# Autodesk Inventor assembly: B_Legs0
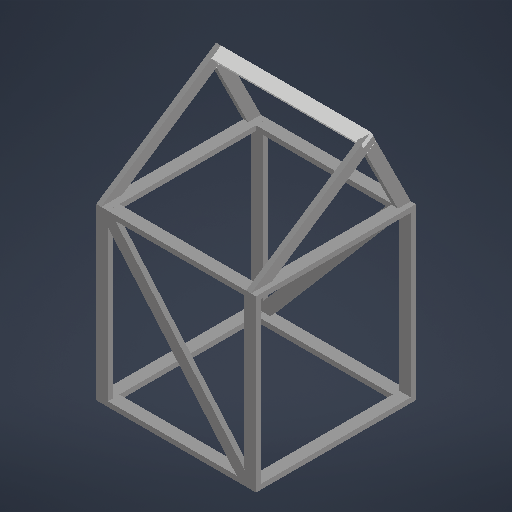
[picture p0: Inventor's stored thumbnail of the model, 512x512]
Saved by Autodesk Inventor 2026 (Build 300175000, 175)
## iProperties
Created: 2024-09-19
Part Number: B_Legs0
Document SubType Name: Assembly
Designer: User
Author: User
## Documents named in this file (8)
- C:\Users\trott\Documents\UofSC-ASME-Tiger-Burn-Design-2025\CAD\Legs\Back Leg\B_Leg.iam
- C:\Users\trott\Documents\UofSC-ASME-Tiger-Burn-Design-2025\CAD\Legs\Back Leg\2x4x96.ipt
- C:\Users\trott\Documents\UofSC-ASME-Tiger-Burn-Design-2025\CAD\Legs\Back Leg\2x4x42.ipt
- C:\Users\trott\Documents\UofSC-ASME-Tiger-Burn-Design-2025\CAD\Legs\Back Leg\2x4x48.ipt
- C:\Users\trott\Documents\UofSC-ASME-Tiger-Burn-Design-2025\CAD\Legs\Back Leg\S_2x4x44.ipt
- C:\Users\trott\Documents\UofSC-ASME-Tiger-Burn-Design-2025\CAD\Legs\Back Leg\2x4x45.ipt
- C:\Users\trott\Documents\UofSC-ASME-Tiger-Burn-Design-2025\CAD\Legs\Back Leg\S_2x4x43.267.ipt
- C:\Users\trott\Documents\UofSC-ASME-Tiger-Burn-Design-2025\CAD\Legs\Back Leg\S_2x4x23.306.ipt
## Components (19 placed, 7 different names)
1. 2x4x96:1 — Flush:1, Flush:2, Flush:3, Flush:4, Flush:5, Flush:8, Mate:3, Flush:10, Flush:12, Flush:13, Flush:14
2. 2x4x96:2 — Mate:1, Flush:1, Flush:2, Flush:3, Mate:2, Flush:6, Flush:7, Mate:5, Flush:9, Flush:11, Flush:15, Flush:16
3. 2x4x42:1 — Flush:4, Flush:5
4. 2x4x42:2 — Mate:2, Flush:6, Flush:7, Mate:4
5. 2x4x48:1 — Flush:8, Flush:13, Flush:14, Mate:7, Flush:17, Flush:20, Flush:29
6. 2x4x48:2 — Mate:5, Flush:15, Flush:16, Mate:6, Flush:18, Flush:19, Flush:27
7. 2x4x48:3 — Mate:4, Flush:9, Flush:11
8. 2x4x48:4 — Mate:3, Flush:10, Flush:12, Mate:13, Flush:28
9. 2x4x96:3 — Mate:7, Flush:17, Flush:20, Mate:8, Mate:9, Flush:23, Flush:24, Flush:29, Flush:33, Mate:19, Flush:34
10. 2x4x96:4 — Mate:6, Flush:18, Flush:19, Flush:21, Flush:22
11. 2x4x42:3 — Mate:8, Flush:21, Flush:22, Mate:12
12. 2x4x42:4 — Mate:9, Flush:23, Flush:24, Mate:18
13. S_2x4x44:1 — Flush:27
14. S_2x4x44:2 — Mate:12, Mate:13, Flush:28
15. 2x4x45:1
16. S_2x4x43.267:1 — Mate:19, Flush:34
17. S_2x4x23.306:1 — Flush:33, Mate:18
18. S_2x4x43.267:2
19. S_2x4x23.306:2
## Relationships (42: Flush 29, Mate 13)
- Mate:1: 2x4x96:2
- Flush:1: 2x4x96:1 ↔ 2x4x96:2
- Flush:2 (1130.3 mm): 2x4x96:1 ↔ 2x4x96:2
- Flush:3: 2x4x96:1 ↔ 2x4x96:2
- Flush:4: 2x4x96:1 ↔ 2x4x42:1
- Flush:5: 2x4x96:1 ↔ 2x4x42:1
- Mate:2: 2x4x96:2 ↔ 2x4x42:2
- Flush:6: 2x4x96:2 ↔ 2x4x42:2
- Flush:7: 2x4x96:2 ↔ 2x4x42:2
- Flush:8: 2x4x96:1 ↔ 2x4x48:1
- Mate:3: 2x4x96:1 ↔ 2x4x48:4
- Mate:4: 2x4x42:2 ↔ 2x4x48:3
- Mate:5: 2x4x96:2 ↔ 2x4x48:2
- Flush:9: 2x4x96:2 ↔ 2x4x48:3
- Flush:10: 2x4x96:1 ↔ 2x4x48:4
- Flush:11: 2x4x96:2 ↔ 2x4x48:3
- Flush:12: 2x4x96:1 ↔ 2x4x48:4
- Flush:13: 2x4x96:1 ↔ 2x4x48:1
- Flush:14: 2x4x96:1 ↔ 2x4x48:1
- Flush:15: 2x4x96:2 ↔ 2x4x48:2
- Flush:16: 2x4x96:2 ↔ 2x4x48:2
- Mate:6: 2x4x48:2 ↔ 2x4x96:4
- Mate:7: 2x4x48:1 ↔ 2x4x96:3
- Flush:17: 2x4x48:1 ↔ 2x4x96:3
- Flush:18: 2x4x48:2 ↔ 2x4x96:4
- Flush:19: 2x4x48:2 ↔ 2x4x96:4
- Flush:20: 2x4x48:1 ↔ 2x4x96:3
- Mate:8: 2x4x96:3 ↔ 2x4x42:3
- Mate:9: 2x4x96:3 ↔ 2x4x42:4
- Flush:21: 2x4x96:4 ↔ 2x4x42:3
- Flush:22: 2x4x96:4 ↔ 2x4x42:3
- Flush:23: 2x4x96:3 ↔ 2x4x42:4
- Flush:24: 2x4x96:3 ↔ 2x4x42:4
- Flush:27: 2x4x48:2 ↔ S_2x4x44:1
- Mate:12: 2x4x42:3 ↔ S_2x4x44:2
- Mate:13: 2x4x48:4 ↔ S_2x4x44:2
- Flush:28: 2x4x48:4 ↔ S_2x4x44:2
- Flush:29: 2x4x48:1 ↔ 2x4x96:3
- Flush:33: 2x4x96:3 ↔ S_2x4x23.306:1
- Mate:18: 2x4x42:4 ↔ S_2x4x23.306:1
- Mate:19: 2x4x96:3 ↔ S_2x4x43.267:1
- Flush:34: 2x4x96:3 ↔ S_2x4x43.267:1
